# Autodesk Inventor assembly: 12in Hex Shaft-ver1-1111-2020
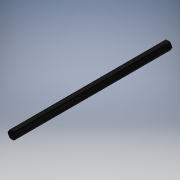
[picture p0: Inventor's stored thumbnail of the model, 180x180]
Saved by Autodesk Inventor 2018 (Build 220112000, 112)
## iProperties
Created: 2020-01-28
Part Number: 12in Hex Shaft-ver1-1111-2020
Document SubType Name: Assembly
Designer: JMHal
Author: JMHal
## Documents named in this file (2)
- F:\GrabCad\2020 Infinite Recharge\Active Climb\Parts\12in Hex Shaft-ver1-1111-2020.iam
- F:\GrabCad\Resources\VEXpro Resources\Shafts\0.5inThunderHexShaft(8)-1111-2016_MIR.ipt
## Components (2 placed, 1 different names)
1. 0.5inThunderHexShaft(8)-1111-2016_MIR:1 — Mate:1, Mate:2, Mate:3
2. 0.5inThunderHexShaft(8)-1111-2016_MIR:2 — Mate:1, Mate:2, Mate:3
## Relationships (3: Mate 3)
- Mate:1: 0.5inThunderHexShaft(8)-1111-2016_MIR:1 ↔ 0.5inThunderHexShaft(8)-1111-2016_MIR:2
- Mate:2: 0.5inThunderHexShaft(8)-1111-2016_MIR:1 ↔ 0.5inThunderHexShaft(8)-1111-2016_MIR:2
- Mate:3: 0.5inThunderHexShaft(8)-1111-2016_MIR:1 ↔ 0.5inThunderHexShaft(8)-1111-2016_MIR:2
